# Autodesk Inventor assembly: trebuchet-assembly
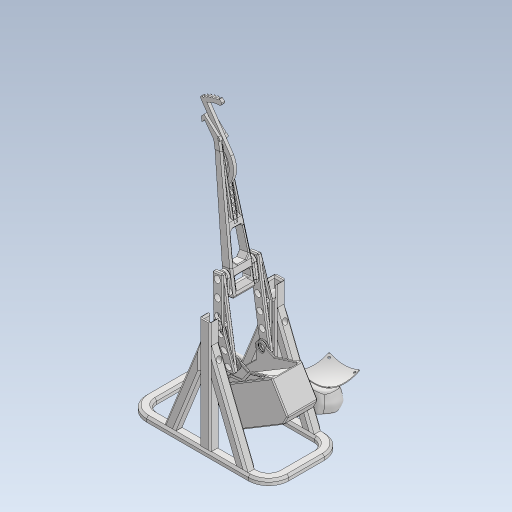
[picture p0: Inventor's stored thumbnail of the model, 512x512]
Saved by Autodesk Inventor 2023 (Build 270158030, 158C)
## iProperties
Created: 2024-12-20
Part Number: trebuchet-assembly
Document SubType Name: Assembly
Designer: Imogen Heard
Author: Imogen Heard
## Documents named in this file (19)
- C:\Users\dheard\Documents\0004-inventor\3D-CAD-main\trebuchet\trebuchet-assembly.iam
- C:\Users\dheard\Documents\0004-inventor\3D-CAD-main\trebuchet\pins.ipt
- C:\Users\dheard\Documents\0004-inventor\3D-CAD-main\trebuchet\bolder.ipt
- C:\Users\dheard\Documents\0004-inventor\3D-CAD-main\trebuchet\sling.ipt
- C:\Users\dheard\Documents\0004-inventor\3D-CAD-main\unicorn-horn\washers.ipt
- C:\Users\dheard\Documents\0004-inventor\3D-CAD-main\trebuchet\V2-baseplate.ipt
- C:\Users\dheard\Documents\0004-inventor\3D-CAD-main\trebuchet\V2-upright-a.ipt
- C:\Users\dheard\Documents\0004-inventor\3D-CAD-main\trebuchet\V2-a-frame.ipt
- C:\Users\dheard\Documents\0004-inventor\3D-CAD-main\trebuchet\V2-pivot-a.ipt
- C:\Users\dheard\Documents\0004-inventor\3D-CAD-main\trebuchet\V2-throw-arm.ipt
- C:\Users\dheard\Documents\0004-inventor\3D-CAD-main\trebuchet\v2-ratchet.ipt
- C:\Users\dheard\Documents\0004-inventor\3D-CAD-main\trebuchet\V2-counterweight.ipt
- C:\Users\dheard\Documents\0004-inventor\3D-CAD-main\trebuchet\V2-pivot-mirror.ipt
- C:\Users\dheard\Documents\0004-inventor\3D-CAD-main\trebuchet\V2-upright-mirror.ipt
- C:\Users\dheard\Documents\0004-inventor\3D-CAD-main\trebuchet\V2-a-frame-B.ipt
- C:\Users\dheard\Documents\0004-inventor\3D-CAD-main\trebuchet\V2-a-frame-C.ipt
- C:\Users\dheard\Documents\0004-inventor\3D-CAD-main\trebuchet\V2-a-frame-D.ipt
- C:\Users\dheard\Documents\0004-inventor\3D-CAD-main\trebuchet\V2-spacer-A.ipt
- C:\Users\dheard\Documents\0004-inventor\3D-CAD-main\trebuchet\V2-spacer-B.ipt
## Components (19 placed, 18 different names)
1. pins:1
2. bolder:1 — Flush:6, Flush:7
3. sling:1 — Flush:6, Flush:7
4. washers:1 — Insert:13
5. V2-baseplate:1
6. V2-upright-a:1 — Rotational:1
7. V2-a-frame:1
8. V2-pivot-a:1 — Rotational:1, Mate:1, Insert:7, Flush:8, Insert:14
9. V2-throw-arm:1 — Insert:8, Insert:9, Mate:2, Insert:10, Insert:11
10. v2-ratchet:1 — Insert:9
11. V2-counterweight:1 — Rotational:2, Insert:13
12. V2-pivot-mirror:1 — Insert:12, Flush:8
13. V2-upright-mirror:1
14. V2-a-frame-B:1
15. V2-a-frame-C:1
16. V2-a-frame-D:1
17. V2-spacer-A:1 — Mate:1, Insert:7, Insert:8, Mate:2
18. V2-spacer-B:1 — Insert:10, Insert:11, Insert:12
19. washers:2 — Rotational:2, Insert:14
## Relationships (15: Insert 8, Flush 3, RevoluteJoint 2, Mate 2)
- Flush:6: bolder:1 ↔ sling:1
- Flush:7: bolder:1 ↔ sling:1
- Rotational:1 [RevoluteJoint] (0.1 mm): V2-upright-a:1 ↔ V2-pivot-a:1
- Mate:1: V2-pivot-a:1 ↔ V2-spacer-A:1
- Insert:7: V2-pivot-a:1 ↔ V2-spacer-A:1
- Insert:8: V2-throw-arm:1 ↔ V2-spacer-A:1
- Insert:9: V2-throw-arm:1 ↔ v2-ratchet:1
- Mate:2: V2-throw-arm:1 ↔ V2-spacer-A:1
- Insert:10: V2-throw-arm:1 ↔ V2-spacer-B:1
- Insert:11: V2-throw-arm:1 ↔ V2-spacer-B:1
- Insert:12: V2-pivot-mirror:1 ↔ V2-spacer-B:1
- Rotational:2 [RevoluteJoint]: V2-counterweight:1 ↔ washers:2
- Insert:13: washers:1 ↔ V2-counterweight:1
- Flush:8: V2-pivot-a:1 ↔ V2-pivot-mirror:1
- Insert:14: V2-pivot-a:1 ↔ washers:2
